# Autodesk Inventor assembly: crane_assembly
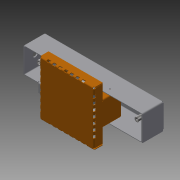
[picture p0: Inventor's stored thumbnail of the model, 180x180]
Saved by Autodesk Inventor 2014 SP2 (Build 180246200, 246)
## iProperties
Created: 2016-05-21
Part Number: crane_assembly
Document SubType Name: Assembly
Designer: cruiser
Author: cruiser
## Documents named in this file (5)
- C:\Users\cruiser\Desktop\models\3d printers\laserresin4\crane_assembly.iam
- C:\Users\cruiser\Desktop\models\3d printers\laserresin4\crane.ipt
- C:\Users\cruiser\Desktop\models\3d printers\laserresin4\bed.ipt
- C:\Users\cruiser\Desktop\models\3d printers\laserresin4\nema17.ipt
- C:\Users\cruiser\Desktop\models\3d printers\laserresin4\lmk8luu.ipt
## Components (5 placed, 4 different names)
1. crane:1 — Mate:1, Mate:2, Mate:3, Mate:4, Mate:5, Mate:6, Mate:7, Mate:8, Mate:9, Mate:10, Mate:11, Mate:12
2. bed:1 — Mate:10, Mate:11, Mate:12
3. nema17:1 — Mate:1, Mate:2, Mate:3
4. lmk8luu:1 — Mate:5, Mate:6, Mate:9
5. lmk8luu:2 — Mate:4, Mate:7, Mate:8
## Relationships (12: Mate 12)
- Mate:1: crane:1 ↔ nema17:1
- Mate:2: crane:1 ↔ nema17:1
- Mate:3: crane:1 ↔ nema17:1
- Mate:4: crane:1 ↔ lmk8luu:2
- Mate:5: crane:1 ↔ lmk8luu:1
- Mate:6: crane:1 ↔ lmk8luu:1
- Mate:7: crane:1 ↔ lmk8luu:2
- Mate:8: crane:1 ↔ lmk8luu:2
- Mate:9: crane:1 ↔ lmk8luu:1
- Mate:10: crane:1 ↔ bed:1
- Mate:11: crane:1 ↔ bed:1
- Mate:12: crane:1 ↔ bed:1
